# Autodesk Inventor assembly: PC Case
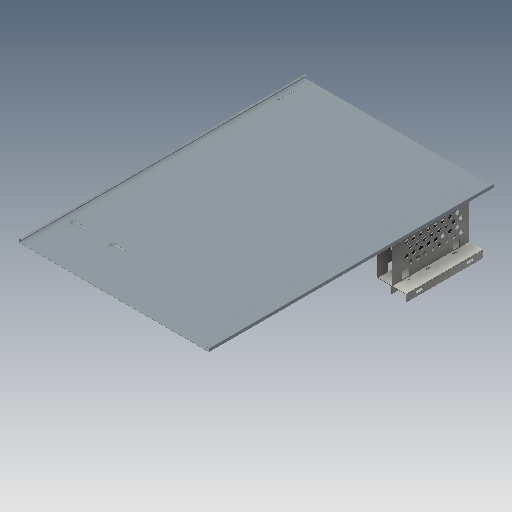
[picture p0: Inventor's stored thumbnail of the model, 512x512]
Saved by Autodesk Inventor 2019.1 (Build 231200000, 200)
## iProperties
Created: 2006-09-21
Part Number: PC Case
Document SubType Name: Assembly
Designer: floress
Description: Controller Assembly
Stock Number: NA
Mass: 341.52 g
Surface Area: 7490.54 cm^2
Volume: 341.52 cm^3
Density: 1 g/cm^3
Author: floress
Title: In House Assembly
Revision Number: A
## Documents named in this file (9)
- C:\Vault Workspace\Process Equipment\Workspace\Supplier Content\Electrical Design\PC Case\PC Case.iam
- C:\Vault Workspace\Process Equipment\Workspace\Supplier Content\Electrical Design\PC Case\Graphic Card Cover.ipt
- C:\Vault Workspace\Process Equipment\Workspace\Supplier Content\Electrical Design\PC Case\Graphic Card Support.ipt
- C:\Vault Workspace\Process Equipment\Workspace\Supplier Content\Electrical Design\PC Case\Module Protector.ipt
- C:\Vault Workspace\Process Equipment\Workspace\Supplier Content\Electrical Design\PC Case\Blank Insert.ipt
- C:\Vault Workspace\Process Equipment\Workspace\Supplier Content\Electrical Design\PC Case\CDROM Bracket 02.ipt
- C:\Vault Workspace\Process Equipment\Workspace\Supplier Content\Electrical Design\PC Case\Hard Drive Bracket.ipt
- C:\Vault Workspace\Process Equipment\Workspace\Supplier Content\Electrical Design\PC Case\Cooling Fan.ipt
- C:\Vault Workspace\Process Equipment\Workspace\Supplier Content\Electrical Design\PC Case\Motherboard Support Wide.ipt
## Components (10 placed, 8 different names)
1. Graphic Card Cover:1 — Mate:30, Mate:31, Mate:32, Mate:51, Mate:52, Mate:54, Mate:58
2. Graphic Card Support:1 — Mate:30, Mate:31, Mate:32, Mate:50, Mate:53
3. Module Protector:1 — Mate:58, Angle:5
4. Blank Insert:1 — Mate:50, Mate:51, Mate:52, Flush:2
5. Blank Insert:2 — Mate:53, Mate:54, Flush:2
6. CDROM Bracket 02:1 — Mate:59
7. Cooling Fan:2
8. Hard Drive Bracket:1 — Mate:36, Mate:37, Mate:38, Flush:3
9. Hard Drive Bracket:2 — Mate:33, Mate:37, Mate:38
10. Motherboard Support Wide:1 — Mate:33, Mate:36, Angle:5, Flush:3, Mate:59
## Relationships (17: Mate 14, Flush 2, Angle 1)
- Mate:30: Graphic Card Cover:1 ↔ Graphic Card Support:1
- Mate:31: Graphic Card Cover:1 ↔ Graphic Card Support:1
- Mate:32: Graphic Card Cover:1 ↔ Graphic Card Support:1
- Mate:33: Hard Drive Bracket:2 ↔ Motherboard Support Wide:1
- Mate:36: Hard Drive Bracket:1 ↔ Motherboard Support Wide:1
- Mate:37: Hard Drive Bracket:1 ↔ Hard Drive Bracket:2
- Mate:38: Hard Drive Bracket:1 ↔ Hard Drive Bracket:2
- Mate:50: Graphic Card Support:1 ↔ Blank Insert:1
- Mate:51: Graphic Card Cover:1 ↔ Blank Insert:1
- Mate:52 (-6.35 mm): Graphic Card Cover:1 ↔ Blank Insert:1
- Mate:53: Graphic Card Support:1 ↔ Blank Insert:2
- Mate:54: Graphic Card Cover:1 ↔ Blank Insert:2
- Flush:2 (21.4884 mm): Blank Insert:1 ↔ Blank Insert:2
- Mate:58: Graphic Card Cover:1 ↔ Module Protector:1
- Angle:5 (0 deg): Module Protector:1 ↔ Motherboard Support Wide:1
- Flush:3: Hard Drive Bracket:1 ↔ Motherboard Support Wide:1
- Mate:59: CDROM Bracket 02:1 ↔ Motherboard Support Wide:1
